# Autodesk Inventor assembly: Push+S+M
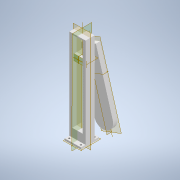
[picture p0: Inventor's stored thumbnail of the model, 180x180]
Saved by Autodesk Inventor 2021 (Build 250183000, 183)
## iProperties
Created: 2022-11-29
Part Number: Push+S+M
Document SubType Name: Assembly
Designer: Elian
Author: Elian
## Documents named in this file (4)
- E:\HTW\5.HTW\Fachübergreifender Projekt\Sprint 1\3d Teile\Push+S+M.iam
- E:\HTW\5.HTW\Fachübergreifender Projekt\Sprint 1\3d Teile\PushSupport.ipt
- E:\HTW\5.HTW\Fachübergreifender Projekt\Sprint 1\3d Teile\Motortest.ipt
- E:\HTW\5.HTW\Fachübergreifender Projekt\Sprint 1\3d Teile\Push.ipt
## Components (3 placed, 3 different names)
1. PushSupport:1 — Passend:1, Passend:3
2. Motortest:1 — Passend:1, Passend:3, Passend:4, Passend:5, Passend:6
3. Push:1 — Passend:4, Passend:5, Passend:6
## Relationships (5: Mate 5)
- Passend:1 [Mate]: PushSupport:1 ↔ Motortest:1
- Passend:3 [Mate]: PushSupport:1 ↔ Motortest:1
- Passend:4 [Mate]: Motortest:1 ↔ Push:1
- Passend:5 [Mate]: Motortest:1 ↔ Push:1
- Passend:6 [Mate]: Motortest:1 ↔ Push:1
